# Autodesk Inventor assembly: OZZ-FullAssembly
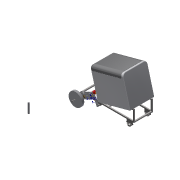
[picture p0: Inventor's stored thumbnail of the model, 180x180]
Saved by Autodesk Inventor 2019.4 (Build 234330000, 330)
## iProperties
Created: 2020-02-15
Part Number: OZZ-FullAssembly
Document SubType Name: Assembly
Designer: Lord of Xy
Mass: 3985.67 g
Surface Area: 2674.25 cm^2
Volume: 722.296 cm^3
Density: 5.51805 g/cm^3
Author: Lord of Xy
## iProperties of the stored document Fridge-Full.iam
Created: 2020-02-07
Part Number: Fridge-Full
Document SubType Name: Assembly
Designer: Simon
Sending System: Autodesk Inventor 2020
Author: Simon
## iProperties of the stored document Fridge-Body.ipt
Created: 2020-02-06
Part Number: Fridge-Body
Material: Generic
Document SubType Name: Modeling
Designer: Simon
Density: 1 g/cm^3
Appearance: Default
Sending System: Autodesk Inventor 2020
Author: Simon
## iProperties of the stored document Fridge-Door.ipt
Created: 2020-02-06
Part Number: Fridge-Door
Material: Generic
Document SubType Name: Modeling
Designer: Simon
Density: 1 g/cm^3
Appearance: Default
Sending System: Autodesk Inventor 2020
Author: Simon
## Documents named in this file (18)
- **C:\Users\Lord of Xy\Documents\Inventor\Ozzie\OZZ-FullAssembly.iam*LocalDocs*xJ0kadk1j5ppiezse1tzzuaseJc*Fridge-Full.iam
- **C:\Users\Lord of Xy\Documents\Inventor\Ozzie\OZZ-FullAssembly.iam*LocalDocs*xG3b0axdiMcbdeqk1Wlaqnusx3h*Fridge-Body.ipt
- **C:\Users\Lord of Xy\Documents\Inventor\Ozzie\OZZ-FullAssembly.iam*LocalDocs*xYy1makrk0ctlemkyH0xyib5p4b*Fridge-Door.ipt
- C:\Users\Lord of Xy\Documents\Inventor\Ozzie\OZZ-FullAssembly.iam
- C:\Users\Lord of Xy\Documents\Inventor\Ozzie\FR00.iam
- C:\Users\Lord of Xy\Documents\Inventor\Ozzie\Suspension\SUS-Sandwich.iam
- C:\Users\Lord of Xy\Documents\Inventor\Ozzie\1865K300_EASY-ACCESS BASE-MOUNTED SHAFT SUPPORT.ipt
- C:\Users\Lord of Xy\Documents\Inventor\Ozzie\Suspension\SUS-Shaft.ipt
- C:\Users\Lord of Xy\Documents\Inventor\Ozzie\Suspension\SUS-ShockAbsorber.ipt
- C:\Users\Lord of Xy\Documents\Inventor\Ozzie\4170T910_CORROSION-RST GAS SPRING.ipt
- C:\Users\Lord of Xy\Documents\Inventor\Ozzie\4167T120_CORROSION-RST EYELET MOUNTING BRACKET.ipt
- C:\Users\Lord of Xy\Documents\Inventor\Ozzie\Suspension\SUS-FrontWheel.ipt
- C:\Users\Lord of Xy\Documents\Inventor\Ozzie\OZZ-BackCaster.ipt
- C:\Users\Lord of Xy\Documents\Inventor\Ozzie\9307K140_BUNA-N RUBBER PUSH-IN GROMMET.ipt
- C:\Users\Lord of Xy\Documents\Inventor\Ozzie\OZZ-CasterRiserBlock.ipt
- C:\Users\Lord of Xy\Documents\Inventor\Ozzie\Fridge-Full.iam
- C:\Users\Lord of Xy\Documents\Inventor\Ozzie\Fridge-Body.ipt
- C:\Users\Lord of Xy\Documents\Inventor\Ozzie\Fridge-Door.ipt
## Components (19 placed, 12 different names)
1. FR00:1 [sub-assembly] — Insert:1, Insert:2, Insert:3, Insert:4, Insert:5, Insert:6, Mate:7, Angle:1, Mate:8, Flush:2, Insert:10, Insert:11, Insert:16, Insert:17
2. SUS-Sandwich:1 [sub-assembly] — Mate:3, Mate:5, Mate:6, Flush:1, Mate:11
3. 1865K300_EASY-ACCESS BASE-MOUNTED SHAFT SUPPORT:1 — Insert:3, Insert:4, Mate:2
4. 1865K300_EASY-ACCESS BASE-MOUNTED SHAFT SUPPORT:2 — Insert:1, Insert:2
5. SUS-Shaft:1 — Mate:2, Mate:3
6. SUS-ShockAbsorber:1 — Mate:9, Mate:10
7. SUS-ShockAbsorber:2
8. Fridge-Full:1 [sub-assembly] — Mate:7, Angle:1
9. 4170T910_CORROSION-RST GAS SPRING:1 — Insert:5, Insert:6, Mate:10
10. 4167T120_CORROSION-RST EYELET MOUNTING BRACKET:1 — Mate:5, Mate:6, Flush:1, Mate:9
11. SUS-FrontWheel:1 — Mate:11
12. OZZ-BackCaster:1 — Insert:7, Insert:8
13. OZZ-BackCaster:2 — Insert:12, Insert:13
14. 9307K140_BUNA-N RUBBER PUSH-IN GROMMET:1 — Insert:7, Insert:9
15. OZZ-CasterRiserBlock:1 — Insert:9, Mate:12, Insert:10, Insert:11
16. 9307K140_BUNA-N RUBBER PUSH-IN GROMMET:2 — Insert:8, Mate:12
17. OZZ-CasterRiserBlock:2 — Insert:14, Insert:15, Insert:16, Insert:17
18. 9307K140_BUNA-N RUBBER PUSH-IN GROMMET:3 — Insert:13, Insert:14
19. 9307K140_BUNA-N RUBBER PUSH-IN GROMMET:4 — Insert:12, Insert:15
## Relationships (30: Insert 17, Mate 10, Flush 2, Angle 1)
- Insert:1: FR00:1 ↔ 1865K300_EASY-ACCESS BASE-MOUNTED SHAFT SUPPORT:2
- Insert:2: FR00:1 ↔ 1865K300_EASY-ACCESS BASE-MOUNTED SHAFT SUPPORT:2
- Insert:3: FR00:1 ↔ 1865K300_EASY-ACCESS BASE-MOUNTED SHAFT SUPPORT:1
- Insert:4: FR00:1 ↔ 1865K300_EASY-ACCESS BASE-MOUNTED SHAFT SUPPORT:1
- Mate:2: 1865K300_EASY-ACCESS BASE-MOUNTED SHAFT SUPPORT:1 ↔ SUS-Shaft:1
- Mate:3: SUS-Sandwich:1 ↔ SUS-Shaft:1
- Insert:5: FR00:1 ↔ 4170T910_CORROSION-RST GAS SPRING:1
- Insert:6: FR00:1 ↔ 4170T910_CORROSION-RST GAS SPRING:1
- Mate:5: SUS-Sandwich:1 ↔ 4167T120_CORROSION-RST EYELET MOUNTING BRACKET:1
- Mate:6: SUS-Sandwich:1 ↔ 4167T120_CORROSION-RST EYELET MOUNTING BRACKET:1
- Flush:1: SUS-Sandwich:1 ↔ 4167T120_CORROSION-RST EYELET MOUNTING BRACKET:1
- Mate:7: FR00:1 ↔ Fridge-Full:1
- Angle:1 (0 deg): FR00:1 ↔ Fridge-Full:1
- Mate:8: FR00:1
- Flush:2: FR00:1
- Mate:9: SUS-ShockAbsorber:1 ↔ 4167T120_CORROSION-RST EYELET MOUNTING BRACKET:1
- Mate:10: SUS-ShockAbsorber:1 ↔ 4170T910_CORROSION-RST GAS SPRING:1
- Mate:11: SUS-Sandwich:1 ↔ SUS-FrontWheel:1
- Insert:7: OZZ-BackCaster:1 ↔ 9307K140_BUNA-N RUBBER PUSH-IN GROMMET:1
- Insert:8: OZZ-BackCaster:1 ↔ 9307K140_BUNA-N RUBBER PUSH-IN GROMMET:2
- Insert:9: 9307K140_BUNA-N RUBBER PUSH-IN GROMMET:1 ↔ OZZ-CasterRiserBlock:1
- Mate:12: OZZ-CasterRiserBlock:1 ↔ 9307K140_BUNA-N RUBBER PUSH-IN GROMMET:2
- Insert:10: FR00:1 ↔ OZZ-CasterRiserBlock:1
- Insert:11: FR00:1 ↔ OZZ-CasterRiserBlock:1
- Insert:12: OZZ-BackCaster:2 ↔ 9307K140_BUNA-N RUBBER PUSH-IN GROMMET:4
- Insert:13: OZZ-BackCaster:2 ↔ 9307K140_BUNA-N RUBBER PUSH-IN GROMMET:3
- Insert:14: OZZ-CasterRiserBlock:2 ↔ 9307K140_BUNA-N RUBBER PUSH-IN GROMMET:3
- Insert:15: OZZ-CasterRiserBlock:2 ↔ 9307K140_BUNA-N RUBBER PUSH-IN GROMMET:4
- Insert:16: FR00:1 ↔ OZZ-CasterRiserBlock:2
- Insert:17: FR00:1 ↔ OZZ-CasterRiserBlock:2
